# Autodesk Inventor assembly: MTLV-S04
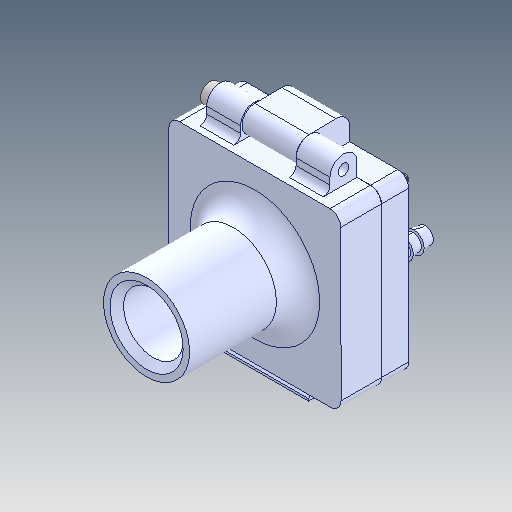
[picture p0: Inventor's stored thumbnail of the model, 512x512]
Saved by Autodesk Inventor 2020 (Build 240168000, 168)
## iProperties
Created: 2020-03-28
Part Number: MTLV-S04
Document SubType Name: Assembly
Designer: John K
Description: AIR OUTLET ASSEMBLY
Author: John K
## Documents named in this file (8)
- C:\GrabCAD\MTL Ventilator Design\MTLV\Subassemblies\MTLV-S04.iam
- C:\GrabCAD\MTL Ventilator Design\MTLV\Manufactured Parts\MTLV-P08.ipt
- C:\GrabCAD\MTL Ventilator Design\MTLV\Manufactured Parts\MTLV-P04.ipt
- C:\GrabCAD\MTL Ventilator Design\MTLV\Manufactured Parts\MTLV-P05.ipt
- C:\GrabCAD\MTL Ventilator Design\MTLV\Commercial Parts\Fasteners\M3x10mm Socket.ipt
- C:\GrabCAD\MTL Ventilator Design\MTLV\Commercial Parts\Fasteners\M4x40mm Socket.ipt
- C:\GrabCAD\MTL Ventilator Design\MTLV\Manufactured Parts\MTLV-M08.ipt
- C:\GrabCAD\MTL Ventilator Design\MTLV\Commercial Parts\Fasteners\M3x6mm Socket.ipt
## Components (12 placed, 7 different names)
1. MTLV-P08:1 — Mate:1, Flush:1, Mate:2, Mate:3, Mate:4, Mate:5, Insert:1, Insert:2, Insert:3, Insert:4, Insert:8
2. MTLV-P04:1 — Mate:1, Flush:1, Mate:5, Insert:5
3. MTLV-P05:1 — Mate:2, Mate:3, Mate:4, Insert:6, Insert:7
4. MTLV-M08:1 — Insert:8, Insert:9
5. M3x6mm Socket:1 — Insert:9
6. M3x10mm Socket:1 — Insert:1
7. M3x10mm Socket:2 — Insert:2
8. M3x10mm Socket:3 — Insert:3
9. M3x10mm Socket:4 — Insert:4
10. M4x40mm Socket:1 — Insert:5
11. M3x10mm Socket:5 — Insert:6
12. M3x10mm Socket:6 — Insert:7
## Relationships (15: Insert 9, Mate 5, Flush 1)
- Mate:1: MTLV-P08:1 ↔ MTLV-P04:1
- Flush:1: MTLV-P08:1 ↔ MTLV-P04:1
- Mate:2: MTLV-P08:1 ↔ MTLV-P05:1
- Mate:3: MTLV-P08:1 ↔ MTLV-P05:1
- Mate:4: MTLV-P08:1 ↔ MTLV-P05:1
- Mate:5: MTLV-P08:1 ↔ MTLV-P04:1
- Insert:1: MTLV-P08:1 ↔ M3x10mm Socket:1
- Insert:2: MTLV-P08:1 ↔ M3x10mm Socket:2
- Insert:3: MTLV-P08:1 ↔ M3x10mm Socket:3
- Insert:4: MTLV-P08:1 ↔ M3x10mm Socket:4
- Insert:5: MTLV-P04:1 ↔ M4x40mm Socket:1
- Insert:6: MTLV-P05:1 ↔ M3x10mm Socket:5
- Insert:7: MTLV-P05:1 ↔ M3x10mm Socket:6
- Insert:8: MTLV-P08:1 ↔ MTLV-M08:1
- Insert:9: MTLV-M08:1 ↔ M3x6mm Socket:1
